# Autodesk Inventor assembly: Fenetre
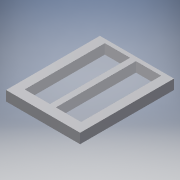
[picture p0: Inventor's stored thumbnail of the model, 180x180]
Saved by Autodesk Inventor 2016 SP1 (Build 200210100, 210)
## iProperties
Created: 2016-10-04
Part Number: Fenetre
Material: Générique
Document SubType Name: Assembly
Designer: dimercur
Author: dimercur
## Documents named in this file (3)
- D:\Users\dimercur\Documents\SVN\projets-gei\Salle 22-24\Fenetre.iam
- D:\Users\dimercur\Documents\SVN\projets-gei\Salle 22-24\Fenetre-Bords.ipt
- D:\Users\dimercur\Documents\SVN\projets-gei\Salle 22-24\Vitre.ipt
## Components (3 placed, 2 different names)
1. Fenetre-Bords:1 — Placage:1, Placage:2, Placage:3, Placage:4
2. Vitre:1 — Placage:1, Placage:2
3. Vitre:2 — Placage:3, Placage:4
## Relationships (4: Mate 4)
- Placage:1 [Mate]: Fenetre-Bords:1 ↔ Vitre:1
- Placage:2 [Mate]: Fenetre-Bords:1 ↔ Vitre:1
- Placage:3 [Mate]: Fenetre-Bords:1 ↔ Vitre:2
- Placage:4 [Mate]: Fenetre-Bords:1 ↔ Vitre:2
